(part 1 of 2)
# Autodesk Inventor assembly: Lift_V2
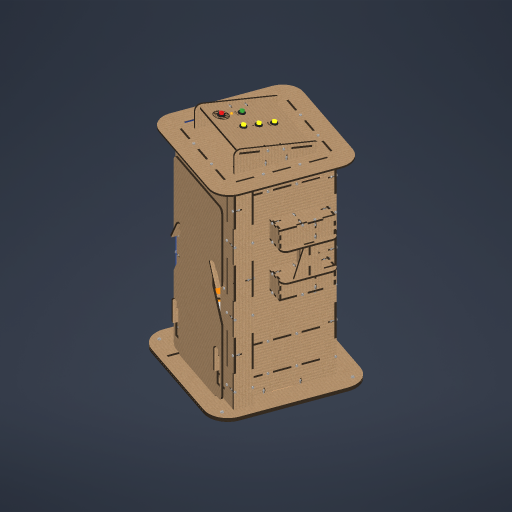
[picture p0: Inventor's stored thumbnail of the model, 512x512]
Saved by Autodesk Inventor 2024.1 (Build 281209000, 209)
## iProperties
Created: 2023-08-03
Part Number: Lift_V2
Document SubType Name: Assembly
Designer: jaege
Mass: 5195.26 g
Surface Area: 20751.9 cm^2
Volume: 3793.96 cm^3
Author: jaege
## Documents named in this file (54)
- C:\Users\jaege\VUB\Schakel_Ind_Elo\Year_1_Both\BA_Thesis\3D_Files\Lift_V2\Lift_V2.iam
- C:\Users\jaege\VUB\Schakel_Ind_Elo\Year_1_Both\BA_Thesis\3D_Files\Lift_V2\Baseplate_V1.ipt
- C:\Users\jaege\VUB\Schakel_Ind_Elo\Year_1_Both\BA_Thesis\3D_Files\Lift_V2\Baseplate_face.ipt
- C:\Users\jaege\VUB\Schakel_Ind_Elo\Year_1_Both\BA_Thesis\3D_Files\Lift_V2\Wall.ipt
- C:\Users\jaege\VUB\Schakel_Ind_Elo\Year_1_Both\BA_Thesis\3D_Files\Lift_V2\Wall_Front.ipt
- C:\Users\jaege\VUB\Schakel_Ind_Elo\Year_1_Both\BA_Thesis\3D_Files\Lift_V2\ISO 7089 - 3 - 140 HV(1).ipt
- C:\Users\jaege\VUB\Schakel_Ind_Elo\Year_1_Both\BA_Thesis\3D_Files\Lift_V2\ISO 1207 - M3 x 12.ipt
- C:\Users\jaege\VUB\Schakel_Ind_Elo\Year_1_Both\BA_Thesis\3D_Files\Lift_V2\ISO 4032 - M3 - ISO.ipt
- C:\Users\jaege\VUB\Schakel_Ind_Elo\Year_1_Both\BA_Thesis\3D_Files\Lift_V2\Wall_rear.ipt
- C:\Users\jaege\VUB\Schakel_Ind_Elo\Year_1_Both\BA_Thesis\3D_Files\Lift_V2\Wall_Left.ipt
- C:\Users\jaege\VUB\Schakel_Ind_Elo\Year_1_Both\BA_Thesis\3D_Files\Lift_V2\Floor.ipt
- C:\Users\jaege\Documents\Inventor\Content Center Files\R2024\en-US\ISO 1207(2)\ISO 1207 - M3 x 12.ipt
- C:\Users\jaege\Documents\Inventor\Content Center Files\R2024\en-US\ISO 4032(2)\ISO 4032 - M3 - ISO.ipt
- C:\Users\jaege\VUB\Schakel_Ind_Elo\Year_1_Both\BA_Thesis\3D_Files\Lift_V2\Floor_Bottom.ipt
- C:\Users\jaege\Documents\Inventor\Content Center Files\R2024\en-US\ISO 1207(2)\ISO 1207 - M3 x 16.ipt
- C:\Users\jaege\VUB\Schakel_Ind_Elo\Year_1_Both\BA_Thesis\3D_Files\Lift_V2\Car_ASM.iam
- C:\Users\jaege\VUB\Schakel_Ind_Elo\Year_1_Both\BA_Thesis\3D_Files\Lift_V2\Floor_Top.ipt
- C:\Users\jaege\VUB\Schakel_Ind_Elo\Year_1_Both\BA_Thesis\3D_Files\Lift_V2\Guide Rod.ipt
- C:\Users\jaege\VUB\Schakel_Ind_Elo\Year_1_Both\BA_Thesis\3D_Files\Lift_V2\Motor24V.ipt
- C:\Users\jaege\VUB\Schakel_Ind_Elo\Year_1_Both\BA_Thesis\3D_Files\Lift_V2\SpindleAdaptor_A.ipt
- C:\Users\jaege\VUB\Schakel_Ind_Elo\Year_1_Both\BA_Thesis\3D_Files\Lift_V2\SpindleAdaptor_B.ipt
- C:\Users\jaege\VUB\Schakel_Ind_Elo\Year_1_Both\BA_Thesis\3D_Files\Lift_V2\Spindle_Rod.ipt
- C:\Users\jaege\Documents\Inventor\Content Center Files\R2024\en-US\ISO 7089\ISO 7089 - 3 - 140 HV(1).ipt
- C:\Users\jaege\Documents\Inventor\Content Center Files\R2024\en-US\ISO 1207(2)\ISO 1207 - M3 x 25.ipt
- C:\Users\jaege\VUB\Schakel_Ind_Elo\Year_1_Both\BA_Thesis\3D_Files\Lift_V2\Cableduct_Cover.ipt
- C:\Users\jaege\VUB\Schakel_Ind_Elo\Year_1_Both\BA_Thesis\3D_Files\Lift_V2\Cableduct_Side.ipt
- C:\Users\jaege\VUB\Schakel_Ind_Elo\Year_1_Both\BA_Thesis\3D_Files\Lift_V2\Cover.ipt
- C:\Users\jaege\VUB\Schakel_Ind_Elo\Year_1_Both\BA_Thesis\3D_Files\Lift_V2\Pannel_Side.ipt
- C:\Users\jaege\VUB\Schakel_Ind_Elo\Year_1_Both\BA_Thesis\3D_Files\Lift_V2\Panel.ipt
- C:\Users\jaege\VUB\Schakel_Ind_Elo\Year_1_Both\BA_Thesis\3D_Files\Lift_V2\Reed_Rail.ipt
- C:\Users\jaege\VUB\Schakel_Ind_Elo\Year_1_Both\BA_Thesis\3D_Files\Lift_V2\SwitchHolder_Top.ipt
- C:\Users\jaege\VUB\Schakel_Ind_Elo\Year_1_Both\BA_Thesis\3D_Files\Lift_V2\SwitchHolder_Bottom.ipt
- C:\Users\jaege\VUB\Schakel_Ind_Elo\Year_1_Both\BA_Thesis\3D_Files\Lift_V2\LimitSwitch_Big.iam
- C:\Users\jaege\VUB\Schakel_Ind_Elo\Year_1_Both\BA_Thesis\3D_Files\Lift_V2\Protector_80x80.ipt
- C:\Users\jaege\VUB\Schakel_Ind_Elo\Year_1_Both\BA_Thesis\3D_Files\Lift_V2\Button_Green.ipt
- C:\Users\jaege\VUB\Schakel_Ind_Elo\Year_1_Both\BA_Thesis\3D_Files\Lift_V2\Button_Red.ipt
- C:\Users\jaege\VUB\Schakel_Ind_Elo\Year_1_Both\BA_Thesis\3D_Files\Lift_V2\Button_Yellow.ipt
- C:\Users\jaege\VUB\Schakel_Ind_Elo\Year_1_Both\BA_Thesis\3D_Files\Lift_V2\LED5mm.ipt
- C:\Users\jaege\VUB\Schakel_Ind_Elo\Year_1_Both\BA_Thesis\3D_Files\Lift_V2\FloorButtonHolder_Back.ipt
- C:\Users\jaege\VUB\Schakel_Ind_Elo\Year_1_Both\BA_Thesis\3D_Files\Lift_V2\FloorButtonHolder_Bottom_A.ipt
- C:\Users\jaege\VUB\Schakel_Ind_Elo\Year_1_Both\BA_Thesis\3D_Files\Lift_V2\FloorButtonHolder_Bottom_B.ipt
- C:\Users\jaege\VUB\Schakel_Ind_Elo\Year_1_Both\BA_Thesis\3D_Files\Lift_V2\FloorButtonHolder_Front.ipt
- C:\Users\jaege\VUB\Schakel_Ind_Elo\Year_1_Both\BA_Thesis\3D_Files\Lift_V2\FloorButtonHolder_Side.ipt
- C:\Users\jaege\VUB\Schakel_Ind_Elo\Year_1_Both\BA_Thesis\3D_Files\Lift_V2\FloorButtonHolder_Top_A.ipt
- C:\Users\jaege\VUB\Schakel_Ind_Elo\Year_1_Both\BA_Thesis\3D_Files\Lift_V2\FloorButtonHolder_Top_B.ipt
- C:\Users\jaege\VUB\Schakel_Ind_Elo\Year_1_Both\BA_Thesis\3D_Files\Lift_V2\LightGateCard.ipt
- C:\Users\jaege\VUB\Schakel_Ind_Elo\Year_1_Both\BA_Thesis\3D_Files\Lift_V2\LightGate_Door.ipt
- C:\Users\jaege\VUB\Schakel_Ind_Elo\Year_1_Both\BA_Thesis\3D_Files\Lift_V2\LightGate_Plate.ipt
- C:\Users\jaege\Documents\Inventor\Content Center Files\R2024\en-US\ISO 1207(2)\ISO 1207 - M3 x 5.ipt
- C:\Users\jaege\VUB\Schakel_Ind_Elo\Year_1_Both\BA_Thesis\3D_Files\Lift_V2\CoverHolder.ipt
- C:\Users\jaege\VUB\Schakel_Ind_Elo\Year_1_Both\BA_Thesis\3D_Files\Lift_V2\Cover_Back.ipt
- C:\Users\jaege\VUB\Schakel_Ind_Elo\Year_1_Both\BA_Thesis\3D_Files\Lift_V2\Spindle_Bearing_Holder.ipt
- C:\Users\jaege\VUB\Schakel_Ind_Elo\Year_1_Both\BA_Thesis\3D_Files\Lift_V2\Lift_V2\Design Accelerator\Bearing1.iam
- C:\Users\jaege\Documents\Inventor\Content Center Files\R2024\en-US\ISO 1207(2)\ISO 1207 - M3 x 10.ipt
## Components (386 placed, 53 different names)
1. Baseplate:1 — Mate:1, Mate:2, Flush:1, Mate:3, Flush:2, Flush:3, Mate:154, Mate:155, Mate:156, Mate:158, Mate:159, Mate:160, Mate:170, Mate:171, Mate:172, Mate:174, Mate:175, Mate:176, Mate:657, Mate:658, Mate:659, Mate:660, Mate:661, Mate:663
2. Baseplate_face:1 — Mate:3, Flush:2, Flush:3, Flush:4, Flush:5, Flush:6, Mate:38, Mate:39, Mate:40, Mate:43, Mate:44, Mate:778, Angle:40
3. Wall:1 — Flush:4, Flush:5, Flush:6, Mate:47, Mate:48, Mate:49, Angle:1, Mate:54, Mate:55, Mate:56, Mate:57, Mate:62, Mate:63, Mate:64, Mate:65, Mate:70, Mate:119, Mate:120, Mate:121, Mate:126, Mate:127, Mate:128, Mate:129, Mate:134, Mate:135, Mate:136, Mate:137, Mate:142, Angle:2, Angle:4, Angle:6, Angle:20, Angle:23, Mate:143, Mate:144, Mate:145, Mate:146, Mate:147, Mate:149, Mate:157, Mate:161, Mate:633, Mate:634, Mate:635, Mate:636, Mate:637, Mate:638, Mate:639, Mate:640, Mate:641, Mate:643, Mate:645, Mate:647, Mate:654, Mate:656, Angle:45, Mate:799, Angle:50, Angle:51, Angle:52, Angle:53
4. Wall_Front:1 — Mate:38, Mate:39, Mate:40, Flush:7, Flush:8, Mate:98, Mate:99, Mate:100, Mate:101, Mate:106, Mate:107, Mate:108, Mate:109, Mate:114, Mate:115, Mate:116, Mate:117, Mate:122, Mate:123, Mate:124, Mate:125, Mate:130, Mate:131, Mate:132, Mate:133, Mate:138, Mate:139, Mate:140, Mate:141, Angle:3, Angle:5, Angle:7, Angle:9, Angle:11, Angle:13, Mate:359, Flush:17, Mate:416, Mate:417, Mate:418, Mate:440, Mate:444, Mate:448, Mate:452, Mate:456, Mate:460, Mate:464, Mate:468, Mate:469, Mate:470, Mate:471, Mate:473, Mate:474, Mate:475, Mate:477, Mate:478, Mate:479, Mate:481, Mate:482, Mate:483, Mate:485, Mate:486, Mate:487, Mate:489, Mate:490, Mate:491, Mate:536, Mate:540, Mate:662, Mate:664, Flush:21, Flush:22, Mate:781, Mate:782, Angle:54, Angle:55, Angle:56, Angle:57
5. Wall_rear:1 — Mate:43, Mate:45, Mate:46, Mate:50, Mate:51, Mate:52, Mate:53, Mate:58, Mate:59, Mate:60, Mate:61, Mate:66, Mate:67, Mate:68, Mate:69, Mate:75, Mate:76, Mate:77, Mate:83, Mate:84, Mate:85, Mate:91, Mate:92, Mate:93, Angle:21, Angle:22, Angle:24, Mate:151, Mate:152, Mate:153, Flush:10, Mate:493, Mate:494, Mate:495, Mate:497, Mate:498, Mate:499, Mate:501, Mate:502, Mate:503, Mate:505, Mate:506, Mate:507, Mate:509, Mate:510, Mate:511, Mate:513, Mate:514, Mate:515, Mate:520, Mate:524, Mate:573, Mate:574, Mate:575, Mate:580, Mate:581, Mate:582, Mate:583, Mate:590, Mate:592, Mate:774, Mate:776, Mate:779, Flush:23, Mate:799, Mate:800, Mate:801, Mate:802, Mate:803, Mate:804, Mate:805, Mate:806, Mate:807, Mate:808, Mate:809, Mate:810, Mate:811, Angle:63, Angle:65, Angle:67, Mate:815, Mate:816, Mate:817, Mate:818, Mate:819, Mate:820, Mate:821, Mate:822, Mate:823, Mate:825, Mate:827, Mate:829
6. Wall_Left:1 — Mate:44, Mate:45, Mate:46, Mate:78, Mate:86, Mate:94, Mate:95, Mate:96, Mate:97, Mate:102, Mate:103, Mate:104, Mate:105, Mate:110, Mate:111, Mate:112, Mate:113, Mate:118, Angle:8, Angle:10, Angle:12, Angle:14, Angle:16, Angle:18, Mate:173, Mate:177, Mate:360, Mate:361, Flush:11, Mate:410, Mate:528, Mate:532, Mate:609, Mate:610, Mate:611, Mate:612, Mate:613, Mate:614, Mate:615, Mate:616, Mate:617, Mate:618, Mate:619, Mate:620, Mate:621, Mate:623, Mate:625, Mate:627, Mate:629, Mate:631, Mate:695, Mate:702, Mate:703, Mate:704, Mate:705, Mate:706, Mate:707, Mate:708, Mate:709, Mate:710, Mate:712, Mate:714, Mate:716, Mate:780, Angle:58, Angle:59
7. Floor:1 — Flush:7, Flush:8, Mate:148, Mate:150, Angle:25, Angle:26, Flush:9, Mate:362, Mate:363, Mate:476, Mate:484, Mate:504, Mate:508, Mate:622, Mate:624, Mate:626, Mate:628, Mate:630, Mate:632, Flush:23
8. Floor_Bottom:1 — Mate:151, Mate:152, Mate:153, Mate:364, Mate:365, Mate:366, Mate:396, Mate:397, Mate:398, Flush:14, Mate:436, Mate:472, Mate:480, Mate:496, Mate:500, Mate:642, Mate:644, Mate:646, Mate:648, Mate:783, Mate:784, Mate:785, Angle:30, Angle:44, Mate:787, Mate:788, Mate:789, Mate:790, Mate:791, Mate:792, Mate:793, Mate:794, Mate:795, Mate:796, Mate:797, Mate:798, Angle:49, Angle:86, Angle:87, Angle:88, Angle:89, Angle:90, Angle:91, Mate:859, Mate:860, Mate:861, Mate:862, Mate:863, Mate:865, Flush:27, Mate:884, Mate:886, Mate:888, Mate:890, Mate:892, Mate:894, Mate:901, Angle:96, Angle:99
9. Car_ASM:1 [sub-assembly] — Mate:367, Mate:409, Mate:415
10. Floor_Top:1 — Mate:359, Mate:360, Mate:361, Mate:399, Mate:400, Mate:488, Mate:492, Mate:512, Mate:516, Mate:786, Mate:847, Mate:848, Mate:849, Mate:850, Mate:851, Mate:852, Mate:853, Mate:855, Mate:857
11. Guide Rod:1 — Flush:9, Mate:436
12. Guide Rod:2 — Mate:363, Mate:364
13. Guide Rod:3 — Mate:362, Mate:365
14. Motor24V:1 — Mate:366, Mate:367, Angle:27, Mate:371
15. SpindleAdaptor_A:1 — Mate:368, Mate:369, Angle:27, Mate:371, Mate:372, Mate:373, Mate:375, Mate:376, Mate:377, Mate:379, Mate:380, Mate:381, Mate:383, Mate:384, Mate:385, Mate:387, Mate:388, Mate:389, Flush:26, Mate:867
16. SpindleAdaptor_B:1 — Mate:368, Mate:369, Mate:374, Mate:378, Mate:382, Mate:386, Mate:390
17. Spindle_Rod:1 — Mate:372, Mate:373, Mate:374
18. Cableduct_Cover:1 — Flush:10, Mate:392, Mate:576, Mate:577, Mate:578, Mate:579, Mate:584, Mate:585, Mate:586, Mate:587, Mate:588, Mate:589, Mate:591, Mate:593, Mate:594, Mate:595, Mate:596, Mate:597, Mate:598, Mate:599, Mate:601, Mate:603, Mate:608, Mate:774, Mate:775, Mate:776, Mate:777, Mate:778, Angle:62, Angle:64, Angle:66
19. Cableduct_Side:1 — Mate:392, Mate:600, Mate:602, Mate:604, Mate:605, Mate:606, Mate:607, Mate:775, Mate:777, Angle:94
20. Cover:1 — Flush:11, Flush:12, Mate:393, Mate:394, Mate:395, Mate:434, Mate:435, Mate:517, Mate:518, Mate:519, Mate:521, Mate:522, Mate:523, Mate:525, Mate:526, Mate:527, Mate:529, Mate:530, Mate:531, Mate:533, Mate:534, Mate:535, Mate:537, Mate:538, Mate:539, Mate:557, Mate:558, Mate:559, Mate:561, Mate:562, Mate:563, Mate:565, Mate:566, Mate:567, Mate:569, Mate:570, Mate:571, Mate:649, Mate:650, Mate:651, Mate:652, Mate:653, Mate:655, Mate:779, Mate:780
21. Pannel_Side:1 — Flush:12, Flush:13, Mate:434, Mate:435, Mate:549, Mate:550, Mate:551, Mate:553, Mate:554, Mate:555, Mate:568, Mate:572, Angle:60, Angle:61
22. Pannel_Side:2 — Mate:393, Mate:394, Mate:395, Mate:432, Mate:433, Mate:541, Mate:542, Mate:543, Mate:545, Mate:546, Mate:547, Mate:560, Mate:564
23. Panel:1 — Flush:13, Mate:420, Mate:421, Mate:422, Mate:423, Mate:424, Mate:425, Mate:426, Mate:427, Mate:428, Mate:429, Mate:430, Mate:431, Mate:432, Mate:433, Mate:544, Mate:548, Mate:552, Mate:556
24. Reed_Rail:1 — Mate:396, Mate:783, Mate:784, Mate:785, Mate:854, Mate:856, Mate:858
25. SwitchHolder_Top:1 — Mate:399, Mate:401, Mate:413, Mate:839, Mate:840, Mate:841, Mate:842, Mate:843, Mate:845
26. SwitchHolder_Bottom:1 — Mate:397, Mate:402, Mate:405, Mate:406, Mate:408, Flush:14, Mate:831, Mate:832, Mate:833, Mate:834, Mate:835, Mate:837, Mate:864, Mate:866, Angle:92
27. SwitchHolder_Top:2 — Mate:400, Mate:401, Mate:411, Mate:412, Mate:414, Flush:15, Flush:16, Mate:844, Mate:846
28. SwitchHolder_Bottom:2 — Mate:398, Mate:402, Mate:407, Mate:410, Flush:15, Flush:16, Mate:836, Mate:838, Angle:93
29. LimitSwitch_Big:1 [sub-assembly] — Mate:405, Mate:406, Mate:407, Mate:408, Mate:409
30. LimitSwitch_Big:2 [sub-assembly] — Mate:411, Mate:412, Mate:413, Mate:414, Mate:415
31. Protector_80x80:1 — Flush:17, Mate:437, Mate:438, Mate:439, Mate:441, Mate:442, Mate:443, Mate:445, Mate:446, Mate:447, Mate:449, Mate:450, Mate:451
32. Protector_80x80:2 — Mate:416, Mate:417, Mate:418, Mate:453, Mate:454, Mate:455, Mate:457, Mate:458, Mate:459, Mate:461, Mate:462, Mate:463, Mate:465, Mate:466, Mate:467
33. Button_Green:1 — Mate:423, Mate:429
34. Button_Yellow:2 — Mate:420, Mate:427
35. Button_Yellow:1 — Mate:422, Mate:428
36. LED5mm:1 — Mate:425, Mate:426
37. Button_Red:2 — Mate:424, Mate:431
38. Button_Yellow:3 — Mate:421, Mate:430
39. CoverHolder:1 — Mate:800, Mate:801, Mate:802, Flush:25, Mate:814, Mate:824, Mate:826, Mate:828, Mate:830, Angle:83
40. CoverHolder:2 — Mate:805, Mate:807, Mate:810, Angle:85
41. CoverHolder:3 — Mate:804, Mate:806, Mate:811, Angle:84
42. CoverHolder:4 — Mate:803, Mate:808, Mate:809, Mate:812, Mate:813
43. Cover_Back:1 — Flush:25, Mate:812, Mate:813, Mate:814
44. Spindle_Bearing_Holder:1 — Flush:26, Flush:27, Mate:868, Mate:869, Mate:872, Mate:874, Mate:876, Mate:878, Mate:880, Mate:882, Mate:895, Mate:896, Mate:897, Mate:898, Mate:899, Mate:900, Mate:901
45. Bearing:1 [sub-assembly] — Mate:867, Mate:868, Mate:869
46. ISO 1207 M3 x 16:1 — Mate:154, Mate:155
47. ISO 1207 M3 x 16:7 — Mate:657, Mate:658
48. ISO 4032 M3:92 — Mate:661, Mate:662, Angle:55
49. ISO 1207 M3 x 16:8 — Mate:659, Mate:660
50. ISO 4032 M3:93 — Mate:663, Mate:664, Angle:54
51. ISO 4032 M3:27 — Mate:156, Mate:157, Angle:50
52. ISO 1207 M3 x 16:2 — Mate:158, Mate:159
53. ISO 4032 M3:28 — Mate:160, Mate:161, Angle:51
54. ISO 1207 M3 x 16:5 — Mate:170, Mate:171
55. ISO 4032 M3:31 — Mate:172, Mate:173
56. ISO 1207 M3 x 16:6 — Mate:174, Mate:175
57. ISO 4032 M3:32 — Mate:176, Mate:177
58. ISO 7089 - 3 - 140 HV(1):1
59. ISO 1207 - M3 x 12:1
60. ISO 7089 - 3 - 140 HV(1):2
61. ISO 4032 - M3 - ISO:1
62. ISO 7089 - 3 - 140 HV(1):3
63. ISO 1207 - M3 x 12:2
64. ISO 7089 - 3 - 140 HV(1):4
65. ISO 4032 - M3 - ISO:2
66. ISO 7089 - 3 - 140 HV(1):5
67. ISO 1207 - M3 x 12:3
68. ISO 7089 - 3 - 140 HV(1):6
69. ISO 4032 - M3 - ISO:3
70. ISO 7089 - 3 - 140 HV(1):7
71. ISO 1207 - M3 x 12:4
72. ISO 7089 - 3 - 140 HV(1):8
73. ISO 4032 - M3 - ISO:4
74. ISO 7089 - 3 - 140 HV(1):9
75. ISO 1207 - M3 x 12:5
76. ISO 7089 - 3 - 140 HV(1):10
77. ISO 4032 - M3 - ISO:5
78. ISO 7089 - 3 - 140 HV(1):11
79. ISO 1207 - M3 x 12:6
80. ISO 7089 - 3 - 140 HV(1):12
81. ISO 4032 - M3 - ISO:6
82. ISO 7089 - 3 - 140 HV(1):13
83. ISO 1207 - M3 x 12:7
84. ISO 7089 - 3 - 140 HV(1):14
85. ISO 4032 - M3 - ISO:7
86. ISO 7089 - 3 - 140 HV(1):15
87. ISO 1207 - M3 x 12:8
88. ISO 7089 - 3 - 140 HV(1):16
89. ISO 4032 - M3 - ISO:8
90. ISO 1207 M3 x 5:1 — Mate:787, Mate:788
91. ISO 1207 M3 x 5:2 — Mate:789, Mate:790
92. ISO 1207 M3 x 5:3 — Mate:791, Mate:792
93. ISO 1207 M3 x 5:4 — Mate:793, Mate:794
94. ISO 1207 M3 x 5:5 — Mate:795, Mate:796
95. ISO 1207 M3 x 5:6 — Mate:797, Mate:798
96. ISO 1207 M3 x 12:76 — Mate:633, Mate:634
97. ISO 4032 M3:86 — Mate:641, Mate:642
98. ISO 1207 M3 x 12:77 — Mate:635, Mate:636
99. ISO 1207 M3 x 12:78 — Mate:637, Mate:638
100. ISO 1207 M3 x 12:79 — Mate:639, Mate:640
101. ISO 4032 M3:87 — Mate:643, Mate:644
102. ISO 4032 M3:88 — Mate:645, Mate:646
103. ISO 4032 M3:89 — Mate:647, Mate:648
104. ISO 1207 M3 x 12:80 — Mate:649, Mate:650
105. ISO 4032 M3:90 — Mate:653, Mate:654, Angle:53
106. ISO 1207 M3 x 12:81 — Mate:651, Mate:652
107. ISO 4032 M3:91 — Mate:655, Mate:656, Angle:52
108. ISO 7089 3:9 — Mate:437, Mate:438, Insert:26
109. ISO 1207 M3 x 12:27 — Insert:26, Mate:781, Angle:36
110. ISO 7089 3:10 — Mate:439, Mate:440, Insert:27
111. ISO 4032 M3:37 — Insert:27, Flush:24, Angle:30, Angle:32, Angle:33
112. ISO 7089 3:11 — Mate:441, Mate:442, Insert:28
113. ISO 1207 M3 x 12:28 — Insert:28, Angle:39, Angle:40
114. ISO 7089 3:12 — Mate:443, Mate:444, Insert:29
115. ISO 4032 M3:38 — Insert:29, Angle:33
116. ISO 7089 3:13 — Mate:445, Mate:446, Insert:30
117. ISO 1207 M3 x 12:29 — Insert:30, Mate:782, Angle:38, Angle:39
118. ISO 7089 3:14 — Mate:447, Mate:448, Insert:31
119. ISO 4032 M3:39 — Insert:31, Angle:34
120. ISO 7089 3:15 — Mate:449, Mate:450, Insert:32
121. ISO 1207 M3 x 12:30 — Insert:32, Angle:36, Angle:37, Angle:38
122. ISO 7089 3:16 — Mate:451, Mate:452, Insert:33
123. ISO 4032 M3:40 — Insert:33, Flush:24, Angle:28, Angle:31, Angle:34
124. ISO 7089 3:17 — Mate:453, Mate:454, Insert:34
125. ISO 1207 M3 x 12:31 — Insert:34
126. ISO 7089 3:18 — Mate:455, Mate:456, Insert:35
127. ISO 4032 M3:41 — Insert:35, Angle:29, Angle:32
128. ISO 7089 3:19 — Mate:457, Mate:458, Insert:36
129. ISO 1207 M3 x 12:32 — Insert:36, Angle:37
130. ISO 7089 3:20 — Mate:459, Mate:460, Insert:37
131. ISO 4032 M3:42 — Insert:37, Angle:28, Angle:29, Angle:31
132. ISO 7089 3:21 — Mate:461, Mate:462, Insert:38
133. ISO 1207 M3 x 12:33 — Insert:38, Angle:35
134. ISO 7089 3:22 — Mate:463, Mate:464, Insert:39
135. ISO 4032 M3:43 — Insert:39
136. ISO 7089 3:23 — Mate:465, Mate:466, Insert:40
137. ISO 1207 M3 x 12:34 — Insert:40, Angle:35
138. ISO 7089 3:24 — Mate:467, Mate:468, Insert:41
139. ISO 4032 M3:44 — Insert:41
140. ISO 1207 M3 x 12:35 — Mate:469, Mate:470
141. ISO 4032 M3:45 — Mate:471, Mate:472, Angle:88
142. ISO 1207 M3 x 12:36 — Mate:473, Mate:474
143. ISO 4032 M3:46 — Mate:475, Mate:476
144. ISO 1207 M3 x 12:37 — Mate:477, Mate:478
145. ISO 4032 M3:47 — Mate:479, Mate:480, Angle:89
146. ISO 1207 M3 x 12:38 — Mate:481, Mate:482
147. ISO 4032 M3:48 — Mate:483, Mate:484
148. ISO 1207 M3 x 12:39 — Mate:485, Mate:486
149. ISO 4032 M3:49 — Mate:487, Mate:488
150. ISO 1207 M3 x 12:40 — Mate:489, Mate:490
151. ISO 4032 M3:50 — Mate:491, Mate:492
152. ISO 1207 M3 x 12:41 — Mate:493, Mate:494
153. ISO 4032 M3:51 — Mate:495, Mate:496, Angle:86
154. ISO 1207 M3 x 12:42 — Mate:497, Mate:498
155. ISO 4032 M3:52 — Mate:499, Mate:500, Angle:87
156. ISO 1207 M3 x 12:43 — Mate:501, Mate:502
157. ISO 4032 M3:53 — Mate:503, Mate:504
158. ISO 1207 M3 x 12:44 — Mate:505, Mate:506
159. ISO 4032 M3:54 — Mate:507, Mate:508
160. ISO 1207 M3 x 12:45 — Mate:509, Mate:510
161. ISO 4032 M3:55 — Mate:511, Mate:512
162. ISO 1207 M3 x 12:46 — Mate:513, Mate:514
163. ISO 4032 M3:56 — Mate:515, Mate:516
164. ISO 1207 M3 x 12:47 — Mate:517, Mate:518
165. ISO 4032 M3:57 — Mate:519, Mate:520
166. ISO 1207 M3 x 12:48 — Mate:521, Mate:522
167. ISO 4032 M3:58 — Mate:523, Mate:524
168. ISO 1207 M3 x 12:49 — Mate:525, Mate:526
169. ISO 4032 M3:59 — Mate:527, Mate:528, Angle:59
170. ISO 1207 M3 x 12:50 — Mate:529, Mate:530
171. ISO 4032 M3:60 — Mate:531, Mate:532, Angle:58
172. ISO 1207 M3 x 12:51 — Mate:533, Mate:534
173. ISO 4032 M3:61 — Mate:535, Mate:536, Angle:56
174. ISO 1207 M3 x 12:52 — Mate:537, Mate:538
175. ISO 4032 M3:62 — Mate:539, Mate:540, Angle:57
176. ISO 1207 M3 x 12:53 — Mate:541, Mate:542
177. ISO 4032 M3:63 — Mate:543, Mate:544
178. ISO 1207 M3 x 12:54 — Mate:545, Mate:546
179. ISO 4032 M3:64 — Mate:547, Mate:548
180. ISO 1207 M3 x 12:55 — Mate:549, Mate:550
181. ISO 4032 M3:65 — Mate:551, Mate:552
182. ISO 1207 M3 x 12:56 — Mate:553, Mate:554
183. ISO 4032 M3:66 — Mate:555, Mate:556
184. ISO 1207 M3 x 12:57 — Mate:557, Mate:558
185. ISO 4032 M3:67 — Mate:559, Mate:560
186. ISO 1207 M3 x 12:58 — Mate:561, Mate:562
187. ISO 4032 M3:68 — Mate:563, Mate:564
188. ISO 1207 M3 x 12:59 — Mate:565, Mate:566
189. ISO 4032 M3:69 — Mate:567, Mate:568, Angle:60
190. ISO 1207 M3 x 12:60 — Mate:569, Mate:570
191. ISO 4032 M3:70 — Mate:571, Mate:572, Angle:61
192. ISO 1207 M3 x 12:61 — Mate:573, Mate:574
193. ISO 4032 M3:71 — Mate:575, Mate:576, Angle:62
194. ISO 1207 M3 x 12:62 — Mate:577, Mate:578
195. ISO 4032 M3:72 — Mate:579, Mate:580, Angle:63
196. ISO 1207 M3 x 12:63 — Mate:581, Mate:582
197. ISO 4032 M3:73 — Mate:583, Mate:584, Angle:66
198. ISO 1207 M3 x 12:64 — Mate:585, Mate:586
199. ISO 4032 M3:74 — Mate:589, Mate:590, Angle:67
200. ISO 1207 M3 x 12:65 — Mate:587, Mate:588
201. ISO 4032 M3:75 — Mate:591, Mate:592, Angle:65
202. ISO 1207 M3 x 12:66 — Mate:593, Mate:594
203. ISO 4032 M3:76 — Mate:599, Mate:600
204. ISO 1207 M3 x 12:67 — Mate:595, Mate:596
205. ISO 1207 M3 x 12:68 — Mate:597, Mate:598
206. ISO 4032 M3:77 — Mate:601, Mate:602, Angle:94
207. ISO 4032 M3:78 — Mate:603, Mate:604
208. ISO 1207 M3 x 12:69 — Mate:605, Mate:606
209. ISO 4032 M3:79 — Mate:607, Mate:608, Angle:64
210. ISO 1207 M3 x 12:70 — Mate:609, Mate:610
211. ISO 4032 M3:80 — Mate:621, Mate:622
212. ISO 1207 M3 x 12:71 — Mate:611, Mate:612
213. ISO 1207 M3 x 12:72 — Mate:613, Mate:614
214. ISO 1207 M3 x 12:73 — Mate:615, Mate:616
215. ISO 1207 M3 x 12:74 — Mate:617, Mate:618
216. ISO 1207 M3 x 12:75 — Mate:619, Mate:620
217. ISO 4032 M3:81 — Mate:623, Mate:624, Mate:786
218. ISO 4032 M3:82 — Mate:625, Mate:626, Angle:91
219. ISO 4032 M3:83 — Mate:627, Mate:628, Angle:90
220. ISO 4032 M3:84 — Mate:629, Mate:630
221. ISO 4032 M3:85 — Mate:631, Mate:632
222. ISO 1207 M3 x 12:1 — Mate:47, Mate:48
223. ISO 4032 M3:1 — Mate:49, Mate:50, Angle:21
224. ISO 1207 M3 x 12:2 — Mate:51, Mate:52
225. ISO 4032 M3:2 — Angle:1, Mate:53, Mate:54
226. ISO 1207 M3 x 12:3 — Mate:55, Mate:56
227. ISO 4032 M3:3 — Mate:57, Mate:58, Angle:22
228. ISO 1207 M3 x 12:4 — Mate:59, Mate:60
229. ISO 4032 M3:4 — Mate:61, Mate:62, Angle:23
230. ISO 1207 M3 x 12:5 — Mate:63, Mate:64
231. ISO 4032 M3:5 — Mate:65, Mate:66, Angle:24
232. ISO 1207 M3 x 12:6 — Mate:67, Mate:68
233. ISO 4032 M3:6 — Mate:69, Mate:70, Angle:20
234. ISO 1207 M3 x 12:8 — Mate:75, Mate:76
235. ISO 4032 M3:8 — Mate:77, Mate:78, Angle:18
236. ISO 1207 M3 x 12:10 — Mate:83, Mate:84
237. ISO 4032 M3:10 — Mate:85, Mate:86, Angle:16
238. ISO 1207 M3 x 12:12 — Mate:91, Mate:92
239. ISO 4032 M3:12 — Mate:93, Mate:94, Angle:14
240. ISO 1207 M3 x 12:13 — Mate:95, Mate:96
241. ISO 4032 M3:13 — Mate:97, Mate:98, Angle:13
242. ISO 1207 M3 x 12:14 — Mate:99, Mate:100
243. ISO 4032 M3:14 — Mate:101, Mate:102, Angle:12
244. ISO 1207 M3 x 12:15 — Mate:103, Mate:104
245. ISO 4032 M3:15 — Mate:105, Mate:106, Angle:11
246. ISO 1207 M3 x 12:16 — Mate:107, Mate:108
247. ISO 4032 M3:16 — Mate:109, Mate:110, Angle:10
248. ISO 1207 M3 x 12:17 — Mate:111, Mate:112
249. ISO 4032 M3:17 — Mate:113, Mate:114, Angle:9
250. ISO 1207 M3 x 12:18 — Mate:115, Mate:116
251. ISO 4032 M3:18 — Mate:117, Mate:118, Angle:8
252. ISO 1207 M3 x 12:19 — Mate:119, Mate:120
253. ISO 4032 M3:19 — Mate:121, Mate:122, Angle:7
254. ISO 1207 M3 x 12:20 — Mate:123, Mate:124
255. ISO 4032 M3:20 — Mate:125, Mate:126, Angle:6
256. ISO 1207 M3 x 12:21 — Mate:127, Mate:128
257. ISO 4032 M3:21 — Mate:129, Mate:130, Angle:5
258. ISO 1207 M3 x 12:22 — Mate:131, Mate:132
259. ISO 4032 M3:22 — Mate:133, Mate:134, Angle:4
260. ISO 1207 M3 x 12:23 — Mate:135, Mate:136
261. ISO 4032 M3:23 — Mate:137, Mate:138, Angle:3
262. ISO 1207 M3 x 12:24 — Mate:139, Mate:140
263. ISO 4032 M3:24 — Mate:141, Mate:142, Angle:2
264. ISO 1207 M3 x 12:25 — Mate:143, Mate:144
265. ISO 4032 M3:25 — Mate:147, Mate:148, Angle:26
266. ISO 1207 M3 x 12:26 — Mate:145, Mate:146
267. ISO 4032 M3:26 — Mate:149, Mate:150, Angle:25
268. ISO 7089 3:1 — Mate:375, Mate:376, Insert:18
269. ISO 1207 M3 x 25:1 — Insert:18, Angle:45, Angle:46
270. ISO 7089 3:2 — Mate:377, Mate:378, Insert:19
271. ISO 4032 M3:33 — Insert:19, Angle:41, Angle:42
272. ISO 7089 3:3 — Mate:379, Mate:380, Insert:20
273. ISO 1207 M3 x 25:2 — Insert:20, Angle:47
274. ISO 7089 3:4 — Mate:381, Mate:382, Insert:21
275. ISO 4032 M3:34 — Insert:21, Angle:42
276. ISO 7089 3:5 — Mate:383, Mate:384, Insert:22
277. ISO 1207 M3 x 25:3 — Insert:22, Angle:47, Angle:48, Angle:49
278. ISO 7089 3:6 — Mate:385, Mate:386, Insert:23
279. ISO 4032 M3:35 — Insert:23, Angle:43
280. ISO 7089 3:7 — Mate:387, Mate:388, Insert:24
281. ISO 1207 M3 x 25:4 — Insert:24, Angle:46, Angle:48
282. ISO 7089 3:8 — Mate:389, Mate:390, Insert:25
283. ISO 4032 M3:36 — Insert:25, Angle:41, Angle:43, Angle:44
284. FloorButtonHolder_Back:1 — Mate:674, Mate:675, Mate:676, Mate:726, Mate:727, Mate:728, Mate:729, Mate:731, Mate:733, Mate:734, Mate:736
285. FloorButtonHolder_Bottom_A:1 — Mate:692, Mate:693, Mate:694, Mate:723, Mate:725, Mate:770, Mate:771, Mate:772, Angle:80, Angle:81, Angle:82
286. FloorButtonHolder_Bottom_B:1 — Mate:665, Mate:666, Mate:667, Mate:668, Mate:669, Mate:670, Mate:675, Mate:676, Mate:677, Flush:18, Mate:678, Mate:681, Mate:762, Mate:763, Mate:764, Angle:78
287. FloorButtonHolder_Front:1 — Mate:665, Mate:666, Mate:667, Mate:672, Mate:673, Flush:22, Mate:697, Mate:699, Mate:742, Mate:743, Mate:745, Mate:746, Mate:747, Mate:749, Mate:750, Mate:754
288. FloorButtonHolder_Side:1 — Mate:668, Mate:669, Mate:670, Mate:671, Mate:720, Mate:724, Mate:761, Mate:765, Angle:74, Angle:75
289. FloorButtonHolder_Top_A:1 — Mate:671, Mate:672, Mate:673, Mate:674, Mate:695, Flush:21, Mate:711, Mate:713, Mate:715, Mate:717, Mate:735, Mate:737, Mate:739, Mate:741, Mate:751, Mate:753, Mate:755, Mate:757, Mate:758, Mate:759, Mate:760, Angle:70, Angle:71, Angle:72, Angle:73
290. FloorButtonHolder_Top_B:1 — Mate:679, Mate:680, Flush:19, Mate:684, Mate:685, Mate:686, Mate:688, Mate:689, Mate:690, Mate:691, Mate:766, Mate:767, Mate:768, Angle:68, Angle:69, Angle:79
291. LightGateCard:1 — Mate:700, Mate:701
292. LightGate_Door:1 — Mate:681, Mate:682, Mate:683, Mate:700, Mate:701
293. LightGate_Plate:1 — Mate:677, Flush:18, Mate:678, Mate:679, Mate:680, Flush:19, Mate:682, Mate:683
294. FloorButtonHolder_Side:2 — Mate:684, Mate:685, Mate:686, Mate:687, Flush:20, Mate:693, Mate:694, Mate:718, Mate:719, Mate:721, Mate:722, Mate:769, Mate:773, Angle:76, Angle:77
295. FloorButtonHolder_Back:2 — Mate:690, Mate:691, Flush:20, Mate:730, Mate:732, Mate:738, Mate:740
296. FloorButtonHolder_Front:2 — Mate:687, Mate:688, Mate:689, Mate:692, Mate:696, Mate:698, Mate:744, Mate:748, Mate:752, Mate:756
297. Button_Yellow:4 — Mate:697, Mate:699
298. Button_Yellow:5 — Mate:696, Mate:698
299. ISO 1207 M3 x 12:100 — Mate:815, Mate:816
300. ISO 4032 M3:112 — Mate:823, Mate:824
301. ISO 1207 M3 x 12:101 — Mate:817, Mate:818
302. ISO 1207 M3 x 12:102 — Mate:819, Mate:820
303. ISO 1207 M3 x 12:103 — Mate:821, Mate:822
304. ISO 4032 M3:113 — Mate:825, Mate:826, Angle:83
305. ISO 4032 M3:114 — Mate:827, Mate:828, Angle:84
306. ISO 4032 M3:115 — Mate:829, Mate:830, Angle:85
307. ISO 1207 M3 x 12:106 — Mate:851, Mate:852
308. ISO 4032 M3:122 — Mate:857, Mate:858
309. ISO 7089 3:25 — Mate:831, Mate:832, Insert:42
310. ISO 1207 M3 x 25:5 — Insert:42
311. ISO 7089 3:26 — Mate:835, Mate:836, Insert:44
312. ISO 4032 M3:116 — Insert:44
313. ISO 7089 3:27 — Mate:833, Mate:834, Insert:43
314. ISO 1207 M3 x 25:6 — Insert:43
315. ISO 7089 3:28 — Mate:837, Mate:838, Insert:45
316. ISO 4032 M3:117 — Insert:45
317. ISO 7089 3:29 — Mate:839, Mate:840, Insert:46
318. ISO 1207 M3 x 25:7 — Insert:46
319. ISO 7089 3:30 — Mate:843, Mate:844, Insert:48
320. ISO 4032 M3:118 — Insert:48
321. ISO 7089 3:31 — Mate:841, Mate:842, Insert:47
322. ISO 1207 M3 x 25:8 — Insert:47
323. ISO 7089 3:32 — Mate:845, Mate:846, Insert:49
324. ISO 4032 M3:119 — Insert:49
325. ISO 1207 M3 x 12:104 — Mate:847, Mate:848
326. ISO 4032 M3:120 — Mate:853, Mate:854
327. ISO 1207 M3 x 12:105 — Mate:849, Mate:850
328. ISO 4032 M3:121 — Mate:855, Mate:856
329. ISO 1207 M3 x 12:107 — Mate:859, Mate:860, Angle:95
330. ISO 4032 M3:123 — Mate:863, Mate:864, Angle:92
331. ISO 1207 M3 x 12:108 — Mate:861, Mate:862, Angle:95, Angle:96
332. ISO 4032 M3:124 — Mate:865, Mate:866, Angle:93
333. ISO 1207 M3 x 10:1 — Mate:872, Mate:897, Mate:902
334. ISO 7089 3:33 — Mate:884, Insert:50
335. ISO 4032 M3:125 — Insert:50, Mate:902, Angle:98, Angle:100
336. ISO 1207 M3 x 10:2 — Mate:874, Mate:895, Mate:903
337. ISO 1207 M3 x 10:3 — Mate:876, Mate:896, Mate:904
338. ISO 1207 M3 x 10:4 — Mate:878, Mate:898, Mate:905
339. ISO 1207 M3 x 10:5 — Mate:880, Mate:900, Mate:907
340. ISO 1207 M3 x 10:6 — Mate:882, Mate:899, Mate:906
341. ISO 7089 3:34 — Mate:886, Insert:51
342. ISO 7089 3:35 — Mate:888, Insert:52
343. ISO 7089 3:36 — Mate:890, Insert:53
344. ISO 7089 3:37 — Mate:892, Insert:54
345. ISO 7089 3:38 — Mate:894, Insert:55
346. ISO 4032 M3:126 — Insert:51, Mate:903, Angle:97, Angle:98, Angle:102
347. ISO 4032 M3:127 — Insert:52, Mate:904, Angle:97, Angle:99
348. ISO 4032 M3:128 — Insert:53, Mate:905, Angle:101
349. ISO 4032 M3:129 — Insert:54, Mate:907, Angle:103
350. ISO 4032 M3:130 — Insert:55, Mate:906, Angle:100, Angle:101, Angle:102, Angle:103
351. ISO 1207 M3 x 12:82 — Mate:702, Mate:703
352. ISO 4032 M3:94 — Mate:710, Mate:711, Angle:71
353. ISO 1207 M3 x 12:83 — Mate:704, Mate:705
354. ISO 1207 M3 x 12:84 — Mate:706, Mate:707
355. ISO 1207 M3 x 12:85 — Mate:708, Mate:709
356. ISO 4032 M3:95 — Mate:712, Mate:713
357. ISO 4032 M3:96 — Mate:714, Mate:715, Angle:69
358. ISO 4032 M3:97 — Mate:716, Mate:717, Angle:81
359. ISO 1207 M3 x 12:86 — Mate:718, Mate:719
360. ISO 4032 M3:98 — Mate:722, Mate:723, Angle:82
361. ISO 1207 M3 x 12:87 — Mate:720, Mate:721
362. ISO 4032 M3:99 — Mate:724, Mate:725, Angle:72
363. ISO 1207 M3 x 12:88 — Mate:726, Mate:727
364. ISO 4032 M3:100 — Mate:734, Mate:735, Angle:70
365. ISO 1207 M3 x 12:89 — Mate:728, Mate:729
366. ISO 1207 M3 x 12:90 — Mate:730, Mate:731
367. ISO 1207 M3 x 12:91 — Mate:732, Mate:733
368. ISO 4032 M3:101 — Mate:736, Mate:737
369. ISO 4032 M3:102 — Mate:738, Mate:739, Angle:68
370. ISO 4032 M3:103 — Mate:740, Mate:741
371. ISO 1207 M3 x 12:92 — Mate:742, Mate:743
372. ISO 4032 M3:104 — Mate:750, Mate:751, Angle:73
373. ISO 1207 M3 x 12:93 — Mate:744, Mate:745
374. ISO 1207 M3 x 12:94 — Mate:746, Mate:747
375. ISO 1207 M3 x 12:95 — Mate:748, Mate:749
376. ISO 4032 M3:105 — Mate:752, Mate:753, Angle:79
377. ISO 4032 M3:106 — Mate:754, Mate:755, Angle:78
378. ISO 4032 M3:107 — Mate:756, Mate:757, Angle:80
379. ISO 1207 M3 x 12:96 — Mate:758, Mate:759
380. ISO 4032 M3:108 — Mate:760, Mate:761, Angle:74
381. ISO 1207 M3 x 12:97 — Mate:762, Mate:763
382. ISO 4032 M3:109 — Mate:764, Mate:765, Angle:75
383. ISO 1207 M3 x 12:98 — Mate:766, Mate:767
384. ISO 4032 M3:110 — Mate:768, Mate:769, Angle:76
385. ISO 1207 M3 x 12:99 — Mate:770, Mate:771
386. ISO 4032 M3:111 — Mate:772, Mate:773, Angle:77
## Relationships (867: Mate 686, Angle 100, Insert 54, Flush 27)
- Mate:1: Baseplate:1
- Mate:2: Baseplate:1
- Flush:1: Baseplate:1
- Mate:3: Baseplate:1 ↔ Baseplate_face:1
- Flush:2: Baseplate:1 ↔ Baseplate_face:1
- Flush:3: Baseplate:1 ↔ Baseplate_face:1
- [Mate]: Baseplate_face:1 ↔ ISO 7089 - 3 - 140 HV(1):1
- [Mate]: Baseplate_face:1 ↔ ISO 7089 - 3 - 140 HV(1):1
- [Insert]: ISO 7089 - 3 - 140 HV(1):1 ↔ ISO 1207 - M3 x 12:1
- [Mate]: Baseplate_face:1 ↔ ISO 7089 - 3 - 140 HV(1):2
- [Mate]: Baseplate:1 ↔ ISO 7089 - 3 - 140 HV(1):2
- [Insert]: ISO 7089 - 3 - 140 HV(1):2 ↔ ISO 4032 - M3 - ISO:1
- [Mate]: Baseplate_face:1 ↔ ISO 7089 - 3 - 140 HV(1):3
- [Mate]: Baseplate_face:1 ↔ ISO 7089 - 3 - 140 HV(1):3
- [Insert]: ISO 7089 - 3 - 140 HV(1):3 ↔ ISO 1207 - M3 x 12:2
- [Mate]: Baseplate_face:1 ↔ ISO 7089 - 3 - 140 HV(1):4
- [Mate]: Baseplate:1 ↔ ISO 7089 - 3 - 140 HV(1):4
- [Insert]: ISO 7089 - 3 - 140 HV(1):4 ↔ ISO 4032 - M3 - ISO:2
- [Mate]: Baseplate_face:1 ↔ ISO 7089 - 3 - 140 HV(1):5
- [Mate]: Baseplate_face:1 ↔ ISO 7089 - 3 - 140 HV(1):5
- [Insert]: ISO 7089 - 3 - 140 HV(1):5 ↔ ISO 1207 - M3 x 12:3
- [Mate]: Baseplate_face:1 ↔ ISO 7089 - 3 - 140 HV(1):6
- [Mate]: Baseplate:1 ↔ ISO 7089 - 3 - 140 HV(1):6
- [Insert]: ISO 7089 - 3 - 140 HV(1):6 ↔ ISO 4032 - M3 - ISO:3
- [Mate]: Baseplate_face:1 ↔ ISO 7089 - 3 - 140 HV(1):7
- [Mate]: Baseplate_face:1 ↔ ISO 7089 - 3 - 140 HV(1):7
- [Insert]: ISO 7089 - 3 - 140 HV(1):7 ↔ ISO 1207 - M3 x 12:4
- [Mate]: Baseplate_face:1 ↔ ISO 7089 - 3 - 140 HV(1):8
- [Mate]: Baseplate:1 ↔ ISO 7089 - 3 - 140 HV(1):8
- [Insert]: ISO 7089 - 3 - 140 HV(1):8 ↔ ISO 4032 - M3 - ISO:4
- [Mate]: Baseplate_face:1 ↔ ISO 7089 - 3 - 140 HV(1):9
- [Mate]: Baseplate_face:1 ↔ ISO 7089 - 3 - 140 HV(1):9
- [Insert]: ISO 7089 - 3 - 140 HV(1):9 ↔ ISO 1207 - M3 x 12:5
- [Mate]: Baseplate_face:1 ↔ ISO 7089 - 3 - 140 HV(1):10
- [Mate]: Baseplate:1 ↔ ISO 7089 - 3 - 140 HV(1):10
- [Insert]: ISO 7089 - 3 - 140 HV(1):10 ↔ ISO 4032 - M3 - ISO:5
- [Mate]: Baseplate_face:1 ↔ ISO 7089 - 3 - 140 HV(1):11
- [Mate]: Baseplate_face:1 ↔ ISO 7089 - 3 - 140 HV(1):11
- [Insert]: ISO 7089 - 3 - 140 HV(1):11 ↔ ISO 1207 - M3 x 12:6
- [Mate]: Baseplate_face:1 ↔ ISO 7089 - 3 - 140 HV(1):12
- [Mate]: Baseplate:1 ↔ ISO 7089 - 3 - 140 HV(1):12
- [Insert]: ISO 7089 - 3 - 140 HV(1):12 ↔ ISO 4032 - M3 - ISO:6
- [Mate]: Baseplate_face:1 ↔ ISO 7089 - 3 - 140 HV(1):13
- [Mate]: Baseplate_face:1 ↔ ISO 7089 - 3 - 140 HV(1):13
- [Insert]: ISO 7089 - 3 - 140 HV(1):13 ↔ ISO 1207 - M3 x 12:7
- [Mate]: Baseplate_face:1 ↔ ISO 7089 - 3 - 140 HV(1):14
- [Mate]: Baseplate:1 ↔ ISO 7089 - 3 - 140 HV(1):14
- [Insert]: ISO 7089 - 3 - 140 HV(1):14 ↔ ISO 4032 - M3 - ISO:7
- [Mate]: Baseplate_face:1 ↔ ISO 7089 - 3 - 140 HV(1):15
- [Mate]: Baseplate_face:1 ↔ ISO 7089 - 3 - 140 HV(1):15
- [Insert]: ISO 7089 - 3 - 140 HV(1):15 ↔ ISO 1207 - M3 x 12:8
- [Mate]: Baseplate_face:1 ↔ ISO 7089 - 3 - 140 HV(1):16
- [Mate]: Baseplate:1 ↔ ISO 7089 - 3 - 140 HV(1):16
- [Insert]: ISO 7089 - 3 - 140 HV(1):16 ↔ ISO 4032 - M3 - ISO:8
- Flush:4: Baseplate_face:1 ↔ Wall:1
- Flush:5: Baseplate_face:1 ↔ Wall:1
- Flush:6: Baseplate_face:1 ↔ Wall:1
- Mate:38: Baseplate_face:1 ↔ Wall_Front:1
- Mate:39: Baseplate_face:1 ↔ Wall_Front:1
- Mate:40: Baseplate_face:1 ↔ Wall_Front:1
- Mate:43: Baseplate_face:1 ↔ Wall_rear:1
- Mate:44: Baseplate_face:1 ↔ Wall_Left:1
- Mate:45: Wall_rear:1 ↔ Wall_Left:1
- Mate:46: Wall_rear:1 ↔ Wall_Left:1
- Flush:7: Wall_Front:1 ↔ Floor:1
- Flush:8: Wall_Front:1 ↔ Floor:1
- Mate:47: Wall:1 ↔ ISO 1207 M3 x 12:1
- Mate:48: Wall:1 ↔ ISO 1207 M3 x 12:1
- Mate:49: Wall:1 ↔ ISO 4032 M3:1
- Mate:50: Wall_rear:1 ↔ ISO 4032 M3:1
- Angle:1 (0 deg): Wall:1 ↔ ISO 4032 M3:2
- Mate:51: Wall_rear:1 ↔ ISO 1207 M3 x 12:2
- Mate:52: Wall_rear:1 ↔ ISO 1207 M3 x 12:2
- Mate:53: Wall_rear:1 ↔ ISO 4032 M3:2
- Mate:54: Wall:1 ↔ ISO 4032 M3:2
- Mate:55: Wall:1 ↔ ISO 1207 M3 x 12:3
- Mate:56: Wall:1 ↔ ISO 1207 M3 x 12:3
- Mate:57: Wall:1 ↔ ISO 4032 M3:3
- Mate:58: Wall_rear:1 ↔ ISO 4032 M3:3
- Mate:59: Wall_rear:1 ↔ ISO 1207 M3 x 12:4
- Mate:60: Wall_rear:1 ↔ ISO 1207 M3 x 12:4
- Mate:61: Wall_rear:1 ↔ ISO 4032 M3:4
- Mate:62: Wall:1 ↔ ISO 4032 M3:4
- Mate:63: Wall:1 ↔ ISO 1207 M3 x 12:5
- Mate:64: Wall:1 ↔ ISO 1207 M3 x 12:5
- Mate:65: Wall:1 ↔ ISO 4032 M3:5
- Mate:66: Wall_rear:1 ↔ ISO 4032 M3:5
- Mate:67: Wall_rear:1 ↔ ISO 1207 M3 x 12:6
- Mate:68: Wall_rear:1 ↔ ISO 1207 M3 x 12:6
- Mate:69: Wall_rear:1 ↔ ISO 4032 M3:6
- Mate:70: Wall:1 ↔ ISO 4032 M3:6
- Mate:75: Wall_rear:1 ↔ ISO 1207 M3 x 12:8
- Mate:76: Wall_rear:1 ↔ ISO 1207 M3 x 12:8
- Mate:77: Wall_rear:1 ↔ ISO 4032 M3:8
- Mate:78: Wall_Left:1 ↔ ISO 4032 M3:8
- Mate:83: Wall_rear:1 ↔ ISO 1207 M3 x 12:10
- Mate:84: Wall_rear:1 ↔ ISO 1207 M3 x 12:10
- Mate:85: Wall_rear:1 ↔ ISO 4032 M3:10
- Mate:86: Wall_Left:1 ↔ ISO 4032 M3:10
- Mate:91: Wall_rear:1 ↔ ISO 1207 M3 x 12:12
- Mate:92: Wall_rear:1 ↔ ISO 1207 M3 x 12:12
- Mate:93: Wall_rear:1 ↔ ISO 4032 M3:12
- Mate:94: Wall_Left:1 ↔ ISO 4032 M3:12
- Mate:95: Wall_Left:1 ↔ ISO 1207 M3 x 12:13
- Mate:96: Wall_Left:1 ↔ ISO 1207 M3 x 12:13
- Mate:97: Wall_Left:1 ↔ ISO 4032 M3:13
- Mate:98: Wall_Front:1 ↔ ISO 4032 M3:13
- Mate:99: Wall_Front:1 ↔ ISO 1207 M3 x 12:14
- Mate:100: Wall_Front:1 ↔ ISO 1207 M3 x 12:14
- Mate:101: Wall_Front:1 ↔ ISO 4032 M3:14
- Mate:102: Wall_Left:1 ↔ ISO 4032 M3:14
- Mate:103: Wall_Left:1 ↔ ISO 1207 M3 x 12:15
- Mate:104: Wall_Left:1 ↔ ISO 1207 M3 x 12:15
- Mate:105: Wall_Left:1 ↔ ISO 4032 M3:15
- Mate:106: Wall_Front:1 ↔ ISO 4032 M3:15
- Mate:107: Wall_Front:1 ↔ ISO 1207 M3 x 12:16
- Mate:108: Wall_Front:1 ↔ ISO 1207 M3 x 12:16
- Mate:109: Wall_Front:1 ↔ ISO 4032 M3:16
- Mate:110: Wall_Left:1 ↔ ISO 4032 M3:16
- Mate:111: Wall_Left:1 ↔ ISO 1207 M3 x 12:17
- Mate:112: Wall_Left:1 ↔ ISO 1207 M3 x 12:17
- Mate:113: Wall_Left:1 ↔ ISO 4032 M3:17
- Mate:114: Wall_Front:1 ↔ ISO 4032 M3:17
- Mate:115: Wall_Front:1 ↔ ISO 1207 M3 x 12:18
- Mate:116: Wall_Front:1 ↔ ISO 1207 M3 x 12:18
- Mate:117: Wall_Front:1 ↔ ISO 4032 M3:18
- Mate:118: Wall_Left:1 ↔ ISO 4032 M3:18
- Mate:119: Wall:1 ↔ ISO 1207 M3 x 12:19
- Mate:120: Wall:1 ↔ ISO 1207 M3 x 12:19
- Mate:121: Wall:1 ↔ ISO 4032 M3:19
- Mate:122: Wall_Front:1 ↔ ISO 4032 M3:19
- Mate:123: Wall_Front:1 ↔ ISO 1207 M3 x 12:20
- Mate:124: Wall_Front:1 ↔ ISO 1207 M3 x 12:20
- Mate:125: Wall_Front:1 ↔ ISO 4032 M3:20
- Mate:126: Wall:1 ↔ ISO 4032 M3:20
- Mate:127: Wall:1 ↔ ISO 1207 M3 x 12:21
- Mate:128: Wall:1 ↔ ISO 1207 M3 x 12:21
- Mate:129: Wall:1 ↔ ISO 4032 M3:21
- Mate:130: Wall_Front:1 ↔ ISO 4032 M3:21
- Mate:131: Wall_Front:1 ↔ ISO 1207 M3 x 12:22
- Mate:132: Wall_Front:1 ↔ ISO 1207 M3 x 12:22
- Mate:133: Wall_Front:1 ↔ ISO 4032 M3:22
- Mate:134: Wall:1 ↔ ISO 4032 M3:22
- Mate:135: Wall:1 ↔ ISO 1207 M3 x 12:23
- Mate:136: Wall:1 ↔ ISO 1207 M3 x 12:23
- Mate:137: Wall:1 ↔ ISO 4032 M3:23
- Mate:138: Wall_Front:1 ↔ ISO 4032 M3:23
- Mate:139: Wall_Front:1 ↔ ISO 1207 M3 x 12:24
- Mate:140: Wall_Front:1 ↔ ISO 1207 M3 x 12:24